# Autodesk Inventor assembly: Assembly2
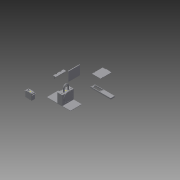
[picture p0: Inventor's stored thumbnail of the model, 180x180]
Saved by Autodesk Inventor 2015 SP2 (Build 190223200, 223)
## iProperties
Created: 2016-09-05
Part Number: Assembly2
Document SubType Name: Assembly
Designer: jm799
Author: jm799
## Documents named in this file (8)
- Z:\My Files\BForcer_modelling\Assembly2.iam
- Z:\My Files\BForcer_modelling\Arduino.ipt
- Z:\My Files\BForcer_modelling\controller_case.ipt
- Z:\My Files\BForcer_modelling\Latch.ipt
- Z:\My Files\BForcer_modelling\Noke.ipt
- Z:\My Files\BForcer_modelling\Noke_holder_latch.ipt
- Z:\My Files\BForcer_modelling\servo.ipt
- Z:\My Files\BForcer_modelling\servo_holder.ipt
## Components (7 placed, 7 different names)
1. Arduino:1
2. controller_case:1
3. Latch:1
4. Noke:1 — Insert:1, Insert:2
5. Noke_holder_latch:1 — Insert:1, Insert:2
6. servo:1
7. servo_holder:1
## Relationships (2: Insert 2)
- Insert:1: Noke:1 ↔ Noke_holder_latch:1
- Insert:2: Noke:1 ↔ Noke_holder_latch:1
